# Autodesk Inventor assembly: 1103 Robot - Master
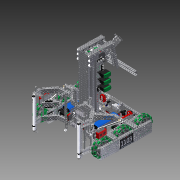
[picture p0: Inventor's stored thumbnail of the model, 180x180]
Saved by Autodesk Inventor 2012 (Build 160160000, 160)
## iProperties
Created: 2011-09-22
Part Number: 1103 Robot - Master
Document SubType Name: Assembly
Designer: Wade
Author: Wade
## Documents named in this file (27)
- C:\Users\Wade\Documents\1103 Robot - CAD Assembly\1103 Robot - Master.iam
- C:\Users\Wade\Documents\1103 Robot - CAD Assembly\1103 Chassis.iam
- C:\Users\Wade\Documents\1103 Robot - CAD Assembly\Left Back Drive Wheel Assembly.iam
- C:\Users\Wade\Documents\1103 Robot - CAD Assembly\Left Drive Wheel Assembly.iam
- C:\Users\Wade\Documents\1103 Robot - CAD Assembly\Drivetrain Motor Sprocket.iam
- C:\Users\Wade\Documents\1103 Robot - CAD Assembly\Drivetrain Encoder Sprocket.iam
- C:\Users\Wade\Documents\1103 Robot - CAD Assembly\Right Back Drive Wheel Assembly.iam
- C:\Users\Wade\Documents\1103 Robot - CAD Assembly\Right Drive Wheel Assembly.iam
- C:\Users\Wade\Documents\1103 Robot - CAD Assembly\1103 Lift - Bottom Tier.iam
- C:\Users\Wade\Documents\1103 Robot - CAD Assembly\1103 Lift - Middle Tier.iam
- C:\Users\Wade\Documents\24C VEX CAD Files\Other Parts\Cylinder, Bi-directional-Parts\Double Acting Cylinder Body.ipt
- C:\Users\Wade\Documents\24C VEX CAD Files\Other Parts\Cylinder, Bi-directional-Parts\Nut 8-32 Hex.ipt
- C:\Users\Wade\Documents\24C VEX CAD Files\Other Parts\Cylinder, Bi-directional-Parts\Double Acting Cylinder Rod.ipt
- C:\Users\Wade\Documents\24C VEX CAD Files\Other Parts\Flow Meter.ipt
- C:\Users\Wade\Documents\24C VEX CAD Files\Other Parts\Fitting for Cylinders.ipt
- C:\Users\Wade\Documents\24C VEX CAD Files\Other Parts\Pneumatic Cylinder Rod Pivot.ipt
- C:\Users\Wade\Documents\1103 Robot - CAD Assembly\1103 Lift -Top Tier.iam
- C:\Users\Wade\Documents\1103 Robot - CAD Assembly\Lift - Top Motor Sprockets.iam
- C:\Users\Wade\Documents\1103 Robot - CAD Assembly\Lift - Bottom Motor Sprocket.iam
- C:\Users\Wade\Documents\1103 Robot - CAD Assembly\Lift - Middle Motor Sprockets.iam
- C:\Users\Wade\Documents\1103 Robot - CAD Assembly\Lift - Main Drive Sprocket.iam
- C:\Users\Wade\Documents\1103 Robot - CAD Assembly\Lift - Bottm Tier Routing Sprocket .iam
- C:\Users\Wade\Documents\1103 Robot - CAD Assembly\Lift - Routing Sprocket.iam
- C:\Users\Wade\Documents\1103 Robot - CAD Assembly\Left Claw.iam
- C:\Users\Wade\Documents\1103 Robot - CAD Assembly\Right Claw.iam
- C:\Users\Wade\Documents\24C VEX CAD Files\Other Parts\Cylinder, Air Push, Spring Return-Parts\Single Acting Cylinder Body.ipt
- C:\Users\Wade\Documents\24C VEX CAD Files\Other Parts\Cylinder, Air Push, Spring Return-Parts\Single Acting Cylinder Rod.ipt
## Components (52 placed, 26 different names)
1. 1103 Chassis:1 [sub-assembly] — Mate:1, Mate:2, Mate:3, Mate:4, Mate:5, Mate:6, Mate:7, Mate:8, Mate:9, Mate:10, Mate:11, Mate:12, Mate:13, Mate:14, Mate:15, Mate:16, Mate:17, Mate:18, Mate:19, Mate:20, Mate:21, Mate:22, Mate:23, Mate:24, Mate:25, Flush:1, Mate:47, Mate:48
2. Left Back Drive Wheel Assembly:1 [sub-assembly] — Mate:1, Mate:2, Rotation:1, Rotation:2, Rotation:3, Rotation:4
3. Left Drive Wheel Assembly:1 [sub-assembly] — Mate:5, Mate:6, Rotation:3
4. Left Drive Wheel Assembly:2 [sub-assembly] — Mate:3, Mate:4, Rotation:4, Rotation:5
5. Drivetrain Motor Sprocket:1 [sub-assembly] — Mate:7, Mate:10, Rotation:5
6. Drivetrain Motor Sprocket:2 [sub-assembly] — Mate:8, Mate:9, Rotation:2
7. Drivetrain Encoder Sprocket:1 [sub-assembly] — Mate:11, Mate:12, Rotation:1
8. Drivetrain Encoder Sprocket:2 [sub-assembly] — Mate:13, Mate:14, Rotation:8
9. Right Back Drive Wheel Assembly:1 [sub-assembly] — Mate:15, Mate:16, Rotation:6, Rotation:8, Rotation:10
10. Right Drive Wheel Assembly:1 [sub-assembly] — Mate:17, Mate:18, Rotation:7
11. Right Drive Wheel Assembly:2 [sub-assembly] — Mate:19, Mate:20, Rotation:9, Rotation:10
12. Drivetrain Motor Sprocket:3 [sub-assembly] — Mate:21, Mate:22, Rotation:9
13. Drivetrain Motor Sprocket:4 [sub-assembly] — Mate:23, Mate:24, Rotation:6, Rotation:7
14. 1103 Lift - Bottom Tier:1 [sub-assembly] — Mate:25, Flush:1, Flush:2, Mate:26, Flush:3, Mate:51, Mate:52, Mate:53, Mate:54, Mate:56, Mate:57, Mate:58, Mate:59, Mate:60, Mate:61, Mate:62, Mate:63, Mate:64, Mate:65, Mate:66, Mate:67, Lift Down
15. 1103 Lift - Middle Tier:1 [sub-assembly] — Flush:2, Mate:26, Flush:3, Flush:8, Mate:55, Lift Movement (Upper Slides), Mate:68, Mate:69, Mate:70, Mate:71
16. Double Acting Cylinder Body:1 — Mate:27, Flush:4, Angle:1, Mate:33, Mate:34, Mate:35, Mate:36, Angle:2, Mate:48
17. Nut 8-32 Hex:1 — Mate:28, Mate:30
18. Double Acting Cylinder Rod:1 — Mate:27, Flush:4, Mate:28, Mate:29, Flush:5, Mate:31
19. Nut 8-32 Hex:2 — Mate:29, Mate:30, Flush:5, Mate:32
20. Flow Meter:1 — Mate:34, Mate:36, Angle:2
21. Fitting for Cylinders:1 — Mate:33, Mate:35
22. Pneumatic Cylinder Rod Pivot:1 — Mate:31, Mate:32, Angle:1, Mate:51, Mate:52
23. Double Acting Cylinder Rod:2 — Mate:37, Lift Tilt Movement, Mate:38, Mate:39, Flush:7, Mate:41
24. Pneumatic Cylinder Rod Pivot:2 — Mate:41, Mate:42, Angle:3, Mate:53, Mate:54
25. Fitting for Cylinders:2 — Mate:43, Mate:45
26. Flow Meter:2 — Mate:44, Mate:46, Angle:4
27. Nut 8-32 Hex:3 — Mate:38, Mate:40, Flush:7, Mate:42, Lift Tilt Up/Forward
28. Nut 8-32 Hex:4 — Mate:39, Mate:40
29. Double Acting Cylinder Body:2 — Mate:37, Lift Tilt Movement, Angle:3, Mate:43, Mate:44, Mate:45, Mate:46, Angle:4, Mate:47, Lift Tilt Up/Forward
30. 1103 Lift -Top Tier:1 [sub-assembly] — Flush:8, Mate:55, Lift Movement (Upper Slides), Rotation/Translation:1, Mate:72, Flush:10, Mate:73, Flush:11, Mate:91, Mate:94, Mate:98, Lift Down
31. Lift - Top Motor Sprockets:1 [sub-assembly] — Mate:56, Mate:57, Rotation:12, Rotation:13
32. Lift - Bottom Motor Sprocket:1 [sub-assembly] — Mate:60, Mate:61, Rotation:11
33. Lift - Middle Motor Sprockets:1 [sub-assembly] — Mate:58, Mate:59, Rotation:11, Rotation:12
34. Lift - Main Drive Sprocket:1 [sub-assembly] — Mate:62, Mate:63, Rotation:13, Rotation/Translation:1, Rotation:15
35. Lift - Bottm Tier Routing Sprocket :1 [sub-assembly] — Mate:66, Mate:67, Rotation:14, Rotation:15
36. Lift - Bottm Tier Routing Sprocket :2 [sub-assembly] — Mate:64, Mate:65, Rotation:14, Rotation:17
37. Lift - Routing Sprocket:1 [sub-assembly] — Mate:68, Mate:69, Rotation:16, Rotation:17
38. Lift - Routing Sprocket:2 [sub-assembly] — Mate:70, Mate:71, Rotation:16
39. Left Claw:1 [sub-assembly] — Mate:73, Flush:11, Mate:95, Mate:96, Mate:98, Rotation:18
40. Right Claw:1 [sub-assembly] — Mate:72, Flush:10, Mate:90, Mate:92, Rotation:18
41. Pneumatic Cylinder Rod Pivot:3 — Mate:80, Angle:6, Mate:90, Mate:92, Mate:108, Mate:109
42. Pneumatic Cylinder Rod Pivot:4 — Mate:81, Angle:5, Mate:95, Mate:96, Mate:104, Mate:105
43. Single Acting Cylinder Body:3 — Mate:74, Mate:82, Mate:84, Angle:6, Mate:91, Right Claw Movement, Right Claw Open
44. Single Acting Cylinder Rod:3 — Mate:74, Mate:80, Right Claw Movement, Right Claw Open, Mate:106, Mate:107, Flush:16
45. Single Acting Cylinder Body:4 — Mate:75, Mate:83, Mate:85, Angle:5, Mate:94, Left Claw Movement, Left Claw Open
46. Single Acting Cylinder Rod:4 — Mate:75, Mate:81, Left Claw Movement, Left Claw Open, Mate:102, Mate:103, Flush:15
47. Fitting for Cylinders:3 — Mate:82, Mate:84
48. Fitting for Cylinders:4 — Mate:83, Mate:85
49. Nut 8-32 Hex:5 — Mate:103, Flush:15, Mate:104
50. Nut 8-32 Hex:6 — Mate:102, Mate:105
51. Nut 8-32 Hex:7 — Mate:106, Mate:108
52. Nut 8-32 Hex:8 — Mate:107, Flush:16, Mate:109
## Relationships (138: Mate 99, RelateRotation 18, Flush 14, Angle 6, RelateRotateTranslate 1)
- Mate:1: 1103 Chassis:1 ↔ Left Back Drive Wheel Assembly:1
- Mate:2: 1103 Chassis:1 ↔ Left Back Drive Wheel Assembly:1
- Mate:3: 1103 Chassis:1 ↔ Left Drive Wheel Assembly:2
- Mate:4: 1103 Chassis:1 ↔ Left Drive Wheel Assembly:2
- Mate:5: 1103 Chassis:1 ↔ Left Drive Wheel Assembly:1
- Mate:6: 1103 Chassis:1 ↔ Left Drive Wheel Assembly:1
- Mate:7: 1103 Chassis:1 ↔ Drivetrain Motor Sprocket:1
- Mate:8: 1103 Chassis:1 ↔ Drivetrain Motor Sprocket:2
- Mate:9: 1103 Chassis:1 ↔ Drivetrain Motor Sprocket:2
- Mate:10: 1103 Chassis:1 ↔ Drivetrain Motor Sprocket:1
- Mate:11: 1103 Chassis:1 ↔ Drivetrain Encoder Sprocket:1
- Mate:12: 1103 Chassis:1 ↔ Drivetrain Encoder Sprocket:1
- Rotation:1 [RelateRotation] (2.4 ul): Left Back Drive Wheel Assembly:1 ↔ Drivetrain Encoder Sprocket:1
- Rotation:2 [RelateRotation] (1 ul): Left Back Drive Wheel Assembly:1 ↔ Drivetrain Motor Sprocket:2
- Rotation:3 [RelateRotation] (1 ul): Left Back Drive Wheel Assembly:1 ↔ Left Drive Wheel Assembly:1
- Rotation:4 [RelateRotation] (1 ul): Left Back Drive Wheel Assembly:1 ↔ Left Drive Wheel Assembly:2
- Rotation:5 [RelateRotation] (1 ul): Left Drive Wheel Assembly:2 ↔ Drivetrain Motor Sprocket:1
- Mate:13: 1103 Chassis:1 ↔ Drivetrain Encoder Sprocket:2
- Mate:14: 1103 Chassis:1 ↔ Drivetrain Encoder Sprocket:2
- Mate:15: 1103 Chassis:1 ↔ Right Back Drive Wheel Assembly:1
- Mate:16: 1103 Chassis:1 ↔ Right Back Drive Wheel Assembly:1
- Mate:17: 1103 Chassis:1 ↔ Right Drive Wheel Assembly:1
- Mate:18: 1103 Chassis:1 ↔ Right Drive Wheel Assembly:1
- Mate:19: 1103 Chassis:1 ↔ Right Drive Wheel Assembly:2
- Mate:20: 1103 Chassis:1 ↔ Right Drive Wheel Assembly:2
- Mate:21: 1103 Chassis:1 ↔ Drivetrain Motor Sprocket:3
- Mate:22: 1103 Chassis:1 ↔ Drivetrain Motor Sprocket:3
- Mate:23: 1103 Chassis:1 ↔ Drivetrain Motor Sprocket:4
- Mate:24: 1103 Chassis:1 ↔ Drivetrain Motor Sprocket:4
- Rotation:6 [RelateRotation] (1 ul): Right Back Drive Wheel Assembly:1 ↔ Drivetrain Motor Sprocket:4
- Rotation:7 [RelateRotation] (1 ul): Right Drive Wheel Assembly:1 ↔ Drivetrain Motor Sprocket:4
- Rotation:8 [RelateRotation] (2.4 ul): Drivetrain Encoder Sprocket:2 ↔ Right Back Drive Wheel Assembly:1
- Rotation:9 [RelateRotation] (1 ul): Right Drive Wheel Assembly:2 ↔ Drivetrain Motor Sprocket:3
- Rotation:10 [RelateRotation] (1 ul): Right Back Drive Wheel Assembly:1 ↔ Right Drive Wheel Assembly:2
- Mate:25: 1103 Chassis:1 ↔ 1103 Lift - Bottom Tier:1
- Flush:1: 1103 Chassis:1 ↔ 1103 Lift - Bottom Tier:1
- Flush:2: 1103 Lift - Bottom Tier:1 ↔ 1103 Lift - Middle Tier:1
- Mate:26 (10.16 mm): 1103 Lift - Bottom Tier:1 ↔ 1103 Lift - Middle Tier:1
- Flush:3: 1103 Lift - Bottom Tier:1 ↔ 1103 Lift - Middle Tier:1
- Mate:27: Double Acting Cylinder Body:1 ↔ Double Acting Cylinder Rod:1
- Flush:4: Double Acting Cylinder Body:1 ↔ Double Acting Cylinder Rod:1
- Mate:28: Nut 8-32 Hex:1 ↔ Double Acting Cylinder Rod:1
- Mate:29: Double Acting Cylinder Rod:1 ↔ Nut 8-32 Hex:2
- Mate:30 (1.1684 mm): Nut 8-32 Hex:1 ↔ Nut 8-32 Hex:2
- Flush:5: Double Acting Cylinder Rod:1 ↔ Nut 8-32 Hex:2
- Mate:31: Double Acting Cylinder Rod:1 ↔ Pneumatic Cylinder Rod Pivot:1
- Mate:32: Nut 8-32 Hex:2 ↔ Pneumatic Cylinder Rod Pivot:1
- Angle:1 (0 deg): Double Acting Cylinder Body:1 ↔ Pneumatic Cylinder Rod Pivot:1
- Mate:33: Double Acting Cylinder Body:1 ↔ Fitting for Cylinders:1
- Mate:34: Double Acting Cylinder Body:1 ↔ Flow Meter:1
- Mate:35: Double Acting Cylinder Body:1 ↔ Fitting for Cylinders:1
- Mate:36: Double Acting Cylinder Body:1 ↔ Flow Meter:1
- Angle:2 (180 deg): Double Acting Cylinder Body:1 ↔ Flow Meter:1
- Mate:37: Double Acting Cylinder Rod:2 ↔ Double Acting Cylinder Body:2
- Lift Tilt Movement [Flush]: Double Acting Cylinder Rod:2 ↔ Double Acting Cylinder Body:2
- Mate:38: Double Acting Cylinder Rod:2 ↔ Nut 8-32 Hex:3
- Mate:39: Double Acting Cylinder Rod:2 ↔ Nut 8-32 Hex:4
- Mate:40 (1.1684 mm): Nut 8-32 Hex:3 ↔ Nut 8-32 Hex:4
- Flush:7: Double Acting Cylinder Rod:2 ↔ Nut 8-32 Hex:3
- Mate:41: Double Acting Cylinder Rod:2 ↔ Pneumatic Cylinder Rod Pivot:2
- Mate:42: Pneumatic Cylinder Rod Pivot:2 ↔ Nut 8-32 Hex:3
- Angle:3 (0 deg): Pneumatic Cylinder Rod Pivot:2 ↔ Double Acting Cylinder Body:2
- Mate:43: Fitting for Cylinders:2 ↔ Double Acting Cylinder Body:2
- Mate:44: Flow Meter:2 ↔ Double Acting Cylinder Body:2
- Mate:45: Fitting for Cylinders:2 ↔ Double Acting Cylinder Body:2
- Mate:46: Flow Meter:2 ↔ Double Acting Cylinder Body:2
- Angle:4 (180 deg): Flow Meter:2 ↔ Double Acting Cylinder Body:2
- Mate:47: 1103 Chassis:1 ↔ Double Acting Cylinder Body:2
- Mate:48: 1103 Chassis:1 ↔ Double Acting Cylinder Body:1
- Mate:51: 1103 Lift - Bottom Tier:1 ↔ Pneumatic Cylinder Rod Pivot:1
- Mate:52: 1103 Lift - Bottom Tier:1 ↔ Pneumatic Cylinder Rod Pivot:1
- Mate:53: 1103 Lift - Bottom Tier:1 ↔ Pneumatic Cylinder Rod Pivot:2
- Mate:54: 1103 Lift - Bottom Tier:1 ↔ Pneumatic Cylinder Rod Pivot:2
- Flush:8: 1103 Lift - Middle Tier:1 ↔ 1103 Lift -Top Tier:1
- Mate:55 (10.16 mm): 1103 Lift - Middle Tier:1 ↔ 1103 Lift -Top Tier:1
- Lift Movement (Upper Slides) [Flush] (-254 mm): 1103 Lift - Middle Tier:1 ↔ 1103 Lift -Top Tier:1
- Mate:56: 1103 Lift - Bottom Tier:1 ↔ Lift - Top Motor Sprockets:1
- Mate:57: 1103 Lift - Bottom Tier:1 ↔ Lift - Top Motor Sprockets:1
- Mate:58: 1103 Lift - Bottom Tier:1 ↔ Lift - Middle Motor Sprockets:1
- Mate:59: 1103 Lift - Bottom Tier:1 ↔ Lift - Middle Motor Sprockets:1
- Mate:60: 1103 Lift - Bottom Tier:1 ↔ Lift - Bottom Motor Sprocket:1
- Mate:61: 1103 Lift - Bottom Tier:1 ↔ Lift - Bottom Motor Sprocket:1
- Rotation:11 [RelateRotation] (1 ul): Lift - Bottom Motor Sprocket:1 ↔ Lift - Middle Motor Sprockets:1
- Rotation:12 [RelateRotation] (1 ul): Lift - Top Motor Sprockets:1 ↔ Lift - Middle Motor Sprockets:1
- Mate:62: 1103 Lift - Bottom Tier:1 ↔ Lift - Main Drive Sprocket:1
- Mate:63: 1103 Lift - Bottom Tier:1 ↔ Lift - Main Drive Sprocket:1
- Rotation:13 [RelateRotation] (0.667 ul): Lift - Top Motor Sprockets:1 ↔ Lift - Main Drive Sprocket:1
- Rotation/Translation:1 [RelateRotateTranslate] (243.84 mm): 1103 Lift -Top Tier:1 ↔ Lift - Main Drive Sprocket:1
- Mate:64: 1103 Lift - Bottom Tier:1 ↔ Lift - Bottm Tier Routing Sprocket :2
- Mate:65: 1103 Lift - Bottom Tier:1 ↔ Lift - Bottm Tier Routing Sprocket :2
- Mate:66: 1103 Lift - Bottom Tier:1 ↔ Lift - Bottm Tier Routing Sprocket :1
- Mate:67: 1103 Lift - Bottom Tier:1 ↔ Lift - Bottm Tier Routing Sprocket :1
- Rotation:14 [RelateRotation] (1 ul): Lift - Bottm Tier Routing Sprocket :1 ↔ Lift - Bottm Tier Routing Sprocket :2
- Rotation:15 [RelateRotation] (0.25 ul): Lift - Main Drive Sprocket:1 ↔ Lift - Bottm Tier Routing Sprocket :1
- Mate:68: 1103 Lift - Middle Tier:1 ↔ Lift - Routing Sprocket:1
- Mate:69: 1103 Lift - Middle Tier:1 ↔ Lift - Routing Sprocket:1
- Mate:70: 1103 Lift - Middle Tier:1 ↔ Lift - Routing Sprocket:2
- Mate:71: 1103 Lift - Middle Tier:1 ↔ Lift - Routing Sprocket:2
- Rotation:16 [RelateRotation] (1 ul): Lift - Routing Sprocket:1 ↔ Lift - Routing Sprocket:2
- Rotation:17 [RelateRotation] (1 ul): Lift - Bottm Tier Routing Sprocket :2 ↔ Lift - Routing Sprocket:1
- Mate:72: 1103 Lift -Top Tier:1 ↔ Right Claw:1
- Flush:10: 1103 Lift -Top Tier:1 ↔ Right Claw:1
- Mate:73: 1103 Lift -Top Tier:1 ↔ Left Claw:1
- Flush:11: 1103 Lift -Top Tier:1 ↔ Left Claw:1
- Mate:74: Single Acting Cylinder Body:3 ↔ Single Acting Cylinder Rod:3
- Mate:75: Single Acting Cylinder Body:4 ↔ Single Acting Cylinder Rod:4
- Mate:80: Pneumatic Cylinder Rod Pivot:3 ↔ Single Acting Cylinder Rod:3
- Mate:81: Pneumatic Cylinder Rod Pivot:4 ↔ Single Acting Cylinder Rod:4
- Mate:82: Single Acting Cylinder Body:3 ↔ Fitting for Cylinders:3
- Mate:83: Single Acting Cylinder Body:4 ↔ Fitting for Cylinders:4
- Mate:84: Single Acting Cylinder Body:3 ↔ Fitting for Cylinders:3
- Mate:85: Single Acting Cylinder Body:4 ↔ Fitting for Cylinders:4
- Angle:5 (0 deg): Pneumatic Cylinder Rod Pivot:4 ↔ Single Acting Cylinder Body:4
- Angle:6 (0 deg): Pneumatic Cylinder Rod Pivot:3 ↔ Single Acting Cylinder Body:3
- Mate:90: Right Claw:1 ↔ Pneumatic Cylinder Rod Pivot:3
- Mate:91: 1103 Lift -Top Tier:1 ↔ Single Acting Cylinder Body:3
- Mate:92: Right Claw:1 ↔ Pneumatic Cylinder Rod Pivot:3
- Right Claw Movement [Mate] (-161.925 mm): Single Acting Cylinder Body:3 ↔ Single Acting Cylinder Rod:3
- Mate:94: 1103 Lift -Top Tier:1 ↔ Single Acting Cylinder Body:4
- Mate:95: Left Claw:1 ↔ Pneumatic Cylinder Rod Pivot:4
- Mate:96: Left Claw:1 ↔ Pneumatic Cylinder Rod Pivot:4
- Left Claw Movement [Mate] (-215.9 mm): Single Acting Cylinder Body:4 ↔ Single Acting Cylinder Rod:4
- Mate:98: 1103 Lift -Top Tier:1 ↔ Left Claw:1
- Lift Tilt Up/Forward [Flush] (-68.58 mm): Nut 8-32 Hex:3 ↔ Double Acting Cylinder Body:2
- Left Claw Open [Mate] (-157.48 mm): Single Acting Cylinder Body:4 ↔ Single Acting Cylinder Rod:4
- Right Claw Open [Mate] (-157.48 mm): Single Acting Cylinder Body:3 ↔ Single Acting Cylinder Rod:3
- Lift Down [Mate]: 1103 Lift - Bottom Tier:1 ↔ 1103 Lift -Top Tier:1
- Rotation:18 [RelateRotation] (1 ul): Left Claw:1 ↔ Right Claw:1
- Mate:102: Single Acting Cylinder Rod:4 ↔ Nut 8-32 Hex:6
- Mate:103: Single Acting Cylinder Rod:4 ↔ Nut 8-32 Hex:5
- Flush:15 (-3.175 mm): Single Acting Cylinder Rod:4 ↔ Nut 8-32 Hex:5
- Mate:104: Pneumatic Cylinder Rod Pivot:4 ↔ Nut 8-32 Hex:5
- Mate:105: Pneumatic Cylinder Rod Pivot:4 ↔ Nut 8-32 Hex:6
- Mate:106: Single Acting Cylinder Rod:3 ↔ Nut 8-32 Hex:7
- Mate:107: Single Acting Cylinder Rod:3 ↔ Nut 8-32 Hex:8
- Flush:16 (3.175 mm): Single Acting Cylinder Rod:3 ↔ Nut 8-32 Hex:8
- Mate:108: Pneumatic Cylinder Rod Pivot:3 ↔ Nut 8-32 Hex:7
- Mate:109: Pneumatic Cylinder Rod Pivot:3 ↔ Nut 8-32 Hex:8
